# Autodesk Inventor assembly: assy_gic_kinematic_2d_robot_arm_MK1_v2
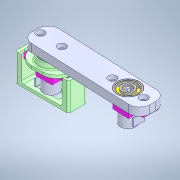
[picture p0: Inventor's stored thumbnail of the model, 180x180]
Saved by Autodesk Inventor 2021 (Build 250183000, 183)
## iProperties
Created: 2021-01-13
Part Number: assy_gic_kinematic_2d_robot_arm_MK1_v2
Document SubType Name: Assembly
Designer: Sam
Sending System: SolidWorks 2020
Last Author: Ben
Last Saved: 2021-01-14
Author: Sam
## Documents named in this file (9)
- D:\OneDrive\MSc Robotics\GIC\RobotKinematics-Remote\3D CAD\Autodesk\15012021\assy_gic_kinematic_2d_robot_arm_MK1_v2.iam
- D:\OneDrive\MSc Robotics\GIC\RobotKinematics-Remote\3D CAD\Autodesk\15012021\2D_robotArm_base_lower_v1.ipt
- D:\OneDrive\MSc Robotics\GIC\RobotKinematics-Remote\3D CAD\Autodesk\15012021\Df_Robot_stepper_FIT0503.ipt
- D:\OneDrive\MSc Robotics\GIC\RobotKinematics-Remote\3D CAD\Autodesk\15012021\base_bearing_holder_v1.ipt
- D:\OneDrive\MSc Robotics\GIC\RobotKinematics-Remote\3D CAD\Autodesk\15012021\608_Z.iam
- D:\OneDrive\MSc Robotics\GIC\RobotKinematics-Remote\3D CAD\Autodesk\15012021\sub_assy_robot_arm_link1.iam
- D:\OneDrive\MSc Robotics\GIC\RobotKinematics-Remote\3D CAD\Autodesk\15012021\DfRobot_stepper_FIT0503_mount_v4.ipt
- C:\Users\Sam\Documents\Inventor\Content Center Files\R2021\en-US\BS 4183(2)\BS 4183 - M3 x 6(1) I.ipt
- C:\Users\Sam\Documents\Inventor\Content Center Files\R2021\en-US\BS 4183(1)\BS 4183 - M3(1).ipt
## Components (10 placed, 8 different names)
1. 2D_robotArm_base_lower_v1:1 — Mate:1, Mate:2, Flush:1
2. DfRobot_stepper_FIT0503_mount_v4:1 — Mate:1, Mate:2, Flush:1, Mate:3, Mate:4, Mate:5, Mate:6, Mate:7, Flush:2, Mate:8, Mate:9, Mate:10, Mate:12
3. Df_Robot_stepper_FIT0503:1 — Mate:4, Mate:5, Mate:6
4. base_bearing_holder_v1:1 — Mate:3, Mate:7, Flush:2, Mate:11, Mate:13
5. 608_Z:1 [sub-assembly]
6. sub_assy_robot_arm_link1:1 [sub-assembly]
7. BS 4183 Cross Recessed Flat Countersunk Head Machine Screw - Metric M3 x 6:1 — Mate:8
8. BS 4183 - Metric M3:1 — Mate:10, Mate:11
9. BS 4183 Cross Recessed Flat Countersunk Head Machine Screw - Metric M3 x 6:2 — Mate:9
10. BS 4183 - Metric M3:2 — Mate:12, Mate:13
## Relationships (15: Mate 13, Flush 2)
- Mate:1: 2D_robotArm_base_lower_v1:1 ↔ DfRobot_stepper_FIT0503_mount_v4:1
- Mate:2: 2D_robotArm_base_lower_v1:1 ↔ DfRobot_stepper_FIT0503_mount_v4:1
- Flush:1: 2D_robotArm_base_lower_v1:1 ↔ DfRobot_stepper_FIT0503_mount_v4:1
- Mate:3: DfRobot_stepper_FIT0503_mount_v4:1 ↔ base_bearing_holder_v1:1
- Mate:4: DfRobot_stepper_FIT0503_mount_v4:1 ↔ Df_Robot_stepper_FIT0503:1
- Mate:5: DfRobot_stepper_FIT0503_mount_v4:1 ↔ Df_Robot_stepper_FIT0503:1
- Mate:6: DfRobot_stepper_FIT0503_mount_v4:1 ↔ Df_Robot_stepper_FIT0503:1
- Mate:7: DfRobot_stepper_FIT0503_mount_v4:1 ↔ base_bearing_holder_v1:1
- Flush:2: DfRobot_stepper_FIT0503_mount_v4:1 ↔ base_bearing_holder_v1:1
- Mate:8: DfRobot_stepper_FIT0503_mount_v4:1 ↔ BS 4183 Cross Recessed Flat Countersunk Head Machine Screw - Metric M3 x 6:1
- Mate:9: DfRobot_stepper_FIT0503_mount_v4:1 ↔ BS 4183 Cross Recessed Flat Countersunk Head Machine Screw - Metric M3 x 6:2
- Mate:10: DfRobot_stepper_FIT0503_mount_v4:1 ↔ BS 4183 - Metric M3:1
- Mate:11: base_bearing_holder_v1:1 ↔ BS 4183 - Metric M3:1
- Mate:12: DfRobot_stepper_FIT0503_mount_v4:1 ↔ BS 4183 - Metric M3:2
- Mate:13: base_bearing_holder_v1:1 ↔ BS 4183 - Metric M3:2
